# Autodesk Inventor assembly: UPPER_LEG_ASM
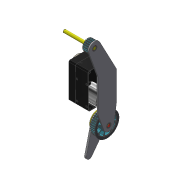
[picture p0: Inventor's stored thumbnail of the model, 180x180]
Saved by Autodesk Inventor 2019.4 (Build 234330000, 330)
## iProperties
Created: 2019-11-12
Part Number: UPPER_LEG_ASM
Material: 一般
Document SubType Name: Assembly
Designer: y6tada
Author: y6tada
## Documents named in this file (13)
- C:\Workspace\Yuni9\Inventor\Asm\UPPER_LEG\UPPER_LEG_ASM.iam
- C:\Workspace\Yuni9\Inventor\Libs\DYNAMIXEL\XM540\XM540_NO_BACK.iam
- C:\Workspace\Yuni9\Inventor\Ref\DDA Series\NMB_A2015\A-2015.iam
- C:\Workspace\Yuni9\Inventor\Asm\UPPER_LEG\ANKLE_DRIVER_LOD.ipt
- C:\Workspace\Yuni9\Inventor\Asm\UPPER_LEG\COXA_PITCH_BEARING_BASE.ipt
- C:\Workspace\Yuni9\Inventor\Asm\UPPER_LEG\UPPER_TIMING_PULLEY_P40.ipt
- C:\Workspace\Yuni9\Inventor\Asm\UPPER_LEG\UPPER_TIMING_PULLEY_COVER_OUTER.ipt
- C:\Workspace\Yuni9\Inventor\Asm\UPPER_LEG\CB-501.5PC.ipt
- C:\Users\y6tada\Documents\Inventor\Content Center Files\R2019\ja-JP\ISO 7046-1 H(1)\ISO 7046-1 - M2 x 14 - 4.8 - H - ISO.ipt
- C:\Workspace\Yuni9\Inventor\Asm\UPPER_LEG\BELT_SUPPORT_INNER.iam
- C:\Workspace\Yuni9\Inventor\Asm\UPPER_LEG\KNEE_DRIVER_ASM.iam
- C:\Workspace\Yuni9\Inventor\Ref\NSK Bearing\NSK_RB_MF85ZZ\MF85ZZ.iam
- C:\Workspace\Yuni9\Inventor\Asm\UPPER_LEG\UPPER_LEG_OUTER_FRAME.ipt
## Components (15 placed, 12 different names)
1. XM540_NO_BACK:1 [sub-assembly] — フラッシュ:2, メイト:30
2. A-2015:1 [sub-assembly] — メイト:1, メイト:5
3. ANKLE_DRIVER_LOD:1 — メイト:3, メイト:9
4. COXA_PITCH_BEARING_BASE:1 — メイト:4, メイト:5, メイト:9, メイト:10, メイト:11, メイト:12
5. UPPER_TIMING_PULLEY_P40:1 — メイト:10, メイト:11, メイト:12, フラッシュ:1, メイト:14, メイト:15, メイト:16, メイト:17, メイト:18, メイト:21, メイト:22, メイト:23, メイト:24
6. UPPER_TIMING_PULLEY_COVER_OUTER:1 — フラッシュ:1, メイト:14, メイト:15, メイト:16
7. CB-501.5PC:1 — メイト:17, メイト:18, メイト:25, メイト:26
8. ISO 7046-1 H M2 x 14 - 4.8 - H:1 — メイト:21
9. ISO 7046-1 H M2 x 14 - 4.8 - H:2 — メイト:22
10. ISO 7046-1 H M2 x 14 - 4.8 - H:3 — メイト:23
11. ISO 7046-1 H M2 x 14 - 4.8 - H:4 — メイト:24
12. BELT_SUPPORT_INNER:1 [sub-assembly]
13. KNEE_DRIVER_ASM:1 [sub-assembly] — メイト:29
14. MF85ZZ:1 [sub-assembly] — メイト:25, メイト:26, メイト:28
15. UPPER_LEG_OUTER_FRAME:1 — メイト:27, メイト:28, メイト:29, フラッシュ:2
## Relationships (25: Mate 23, Flush 2)
- メイト:1 [Mate]: A-2015:1
- メイト:3 [Mate]: ANKLE_DRIVER_LOD:1
- メイト:4 [Mate]: COXA_PITCH_BEARING_BASE:1
- メイト:5 [Mate]: A-2015:1 ↔ COXA_PITCH_BEARING_BASE:1
- メイト:9 [Mate] (1 mm): ANKLE_DRIVER_LOD:1 ↔ COXA_PITCH_BEARING_BASE:1
- メイト:10 [Mate]: COXA_PITCH_BEARING_BASE:1 ↔ UPPER_TIMING_PULLEY_P40:1
- メイト:11 [Mate]: COXA_PITCH_BEARING_BASE:1 ↔ UPPER_TIMING_PULLEY_P40:1
- メイト:12 [Mate]: COXA_PITCH_BEARING_BASE:1 ↔ UPPER_TIMING_PULLEY_P40:1
- フラッシュ:1 [Flush]: UPPER_TIMING_PULLEY_P40:1 ↔ UPPER_TIMING_PULLEY_COVER_OUTER:1
- メイト:14 [Mate]: UPPER_TIMING_PULLEY_P40:1 ↔ UPPER_TIMING_PULLEY_COVER_OUTER:1
- メイト:15 [Mate]: UPPER_TIMING_PULLEY_P40:1 ↔ UPPER_TIMING_PULLEY_COVER_OUTER:1
- メイト:16 [Mate]: UPPER_TIMING_PULLEY_P40:1 ↔ UPPER_TIMING_PULLEY_COVER_OUTER:1
- メイト:17 [Mate]: UPPER_TIMING_PULLEY_P40:1 ↔ CB-501.5PC:1
- メイト:18 [Mate]: UPPER_TIMING_PULLEY_P40:1 ↔ CB-501.5PC:1
- メイト:21 [Mate]: UPPER_TIMING_PULLEY_P40:1 ↔ ISO 7046-1 H M2 x 14 - 4.8 - H:1
- メイト:22 [Mate]: UPPER_TIMING_PULLEY_P40:1 ↔ ISO 7046-1 H M2 x 14 - 4.8 - H:2
- メイト:23 [Mate]: UPPER_TIMING_PULLEY_P40:1 ↔ ISO 7046-1 H M2 x 14 - 4.8 - H:3
- メイト:24 [Mate]: UPPER_TIMING_PULLEY_P40:1 ↔ ISO 7046-1 H M2 x 14 - 4.8 - H:4
- メイト:25 [Mate]: CB-501.5PC:1 ↔ MF85ZZ:1
- メイト:26 [Mate]: CB-501.5PC:1 ↔ MF85ZZ:1
- メイト:27 [Mate]: UPPER_LEG_OUTER_FRAME:1
- メイト:28 [Mate]: MF85ZZ:1 ↔ UPPER_LEG_OUTER_FRAME:1
- メイト:29 [Mate]: KNEE_DRIVER_ASM:1 ↔ UPPER_LEG_OUTER_FRAME:1
- フラッシュ:2 [Flush] (-44 mm): XM540_NO_BACK:1 ↔ UPPER_LEG_OUTER_FRAME:1
- メイト:30 [Mate]: XM540_NO_BACK:1
